# Autodesk Inventor assembly: TR2 Visual Assembly
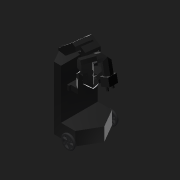
[picture p0: Inventor's stored thumbnail of the model, 180x180]
Saved by Autodesk Inventor 2017 (Build 210142000, 142)
## iProperties
Created: 2019-08-03
Part Number: TR2 Visual Assembly
Document SubType Name: Assembly
Designer: Dell
Author: Dell
## Documents named in this file (12)
- C:\Users\Dell\Documents\GitHub\tr2_essentials\tr2_description\meshes\Visual Assembly\TR2 Visual Assembly.iam
- C:\Users\Dell\Documents\GitHub\tr2_essentials\tr2_description\meshes\Visual Assembly\body.ipt
- C:\Users\Dell\Documents\GitHub\tr2_essentials\tr2_description\meshes\Visual Assembly\link_a0.ipt
- C:\Users\Dell\Documents\GitHub\tr2_essentials\tr2_description\meshes\Visual Assembly\link_a1.ipt
- C:\Users\Dell\Documents\GitHub\tr2_essentials\tr2_description\meshes\Visual Assembly\link_a2.ipt
- C:\Users\Dell\Documents\GitHub\tr2_essentials\tr2_description\meshes\Visual Assembly\link_g0.ipt
- C:\Users\Dell\Documents\GitHub\tr2_essentials\tr2_description\meshes\Visual Assembly\link_g1.ipt
- C:\Users\Dell\Documents\GitHub\tr2_essentials\tr2_description\meshes\Visual Assembly\link_b1.ipt
- C:\Users\Dell\Documents\GitHub\tr2_essentials\tr2_description\meshes\Visual Assembly\link_b2.ipt
- C:\Users\Dell\Documents\GitHub\tr2_essentials\tr2_description\meshes\Visual Assembly\link_b3.ipt
- C:\Users\Dell\Documents\GitHub\tr2_essentials\tr2_description\meshes\Visual Assembly\link_h0.ipt
- C:\Users\Dell\Documents\GitHub\tr2_essentials\tr2_description\meshes\Visual Assembly\link_h1.ipt
## Components (14 placed, 11 different names)
1. body:1 — Mate:1, Mate:2, Mate:17, Mate:18, Mate:19, Mate:20, Mate:21, Mate:22, Mate:25, Mate:26
2. link_a0:1 — Mate:1, Mate:2, Mate:3, Mate:4
3. link_a1:1 — Mate:3, Mate:4, Mate:5, Mate:6
4. link_a2:1 — Mate:5, Mate:6, Mate:7, Mate:8
5. link_a1:2 — Mate:7, Mate:8, Mate:9, Mate:10
6. link_g0:1 — Mate:9, Mate:10, Mate:11, Mate:12, Mate:13, Mate:14, Mate:15, Mate:16
7. link_g1:1 — Mate:11, Mate:12, Mate:16
8. link_g1:2 — Mate:13, Mate:14, Mate:15
9. link_b1:1 — Mate:17, Mate:19
10. link_b1:2 — Mate:18, Mate:20
11. link_b2:1 — Mate:21, Mate:22, Mate:23, Mate:24
12. link_b3:1 — Mate:23, Mate:24
13. link_h0:1 — Mate:25, Mate:26, Mate:27, Mate:28
14. link_h1:1 — Mate:27, Mate:28
## Relationships (28: Mate 28)
- Mate:1: body:1 ↔ link_a0:1
- Mate:2: body:1 ↔ link_a0:1
- Mate:3: link_a0:1 ↔ link_a1:1
- Mate:4: link_a0:1 ↔ link_a1:1
- Mate:5: link_a1:1 ↔ link_a2:1
- Mate:6: link_a1:1 ↔ link_a2:1
- Mate:7: link_a2:1 ↔ link_a1:2
- Mate:8: link_a2:1 ↔ link_a1:2
- Mate:9: link_a1:2 ↔ link_g0:1
- Mate:10: link_a1:2 ↔ link_g0:1
- Mate:11: link_g0:1 ↔ link_g1:1
- Mate:12: link_g0:1 ↔ link_g1:1
- Mate:13: link_g0:1 ↔ link_g1:2
- Mate:14: link_g0:1 ↔ link_g1:2
- Mate:15: link_g0:1 ↔ link_g1:2
- Mate:16: link_g0:1 ↔ link_g1:1
- Mate:17: body:1 ↔ link_b1:1
- Mate:18: body:1 ↔ link_b1:2
- Mate:19 (25 mm): body:1 ↔ link_b1:1
- Mate:20 (25 mm): body:1 ↔ link_b1:2
- Mate:21: body:1 ↔ link_b2:1
- Mate:22: body:1 ↔ link_b2:1
- Mate:23: link_b2:1 ↔ link_b3:1
- Mate:24 (3.7 mm): link_b2:1 ↔ link_b3:1
- Mate:25: body:1 ↔ link_h0:1
- Mate:26: body:1 ↔ link_h0:1
- Mate:27: link_h0:1 ↔ link_h1:1
- Mate:28: link_h0:1 ↔ link_h1:1
